# Autodesk Inventor assembly: Assembly1
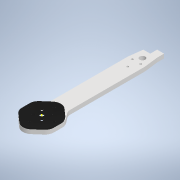
[picture p0: Inventor's stored thumbnail of the model, 180x180]
Saved by Autodesk Inventor 2020 (Build 240168000, 168)
## iProperties
Created: 2021-11-30
Part Number: Assembly1
Document SubType Name: Assembly
Designer: Steven
Author: Steven
## Documents named in this file (3)
- X:\fpv drone stuff\Street league\prig git files\Assembly1.iam
- X:\fpv drone stuff\3d prints\Tx16s\mod arms.ipt
- X:\fpv drone stuff\Street league\prig git files\mod arm plate.ipt
## Components (2 placed, 2 different names)
1. mod arms:1 — Mate:1, Flush:1, Flush:2
2. mod arm plate:1 — Mate:1, Flush:1, Flush:2
## Relationships (3: Flush 2, Mate 1)
- Mate:1: mod arms:1 ↔ mod arm plate:1
- Flush:1: mod arms:1 ↔ mod arm plate:1
- Flush:2: mod arms:1 ↔ mod arm plate:1
